# Autodesk Inventor assembly: Printer Assembly
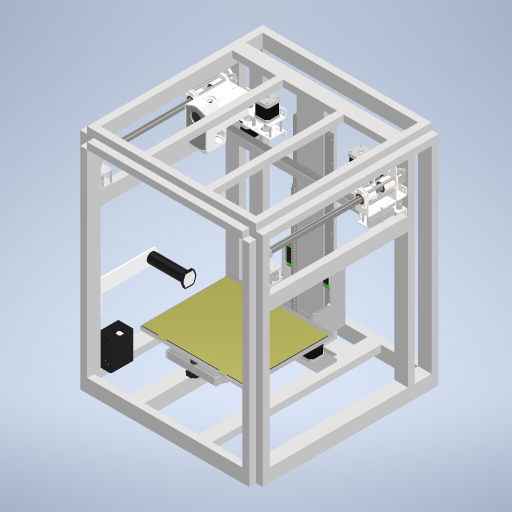
[picture p0: Inventor's stored thumbnail of the model, 512x512]
Saved by Autodesk Inventor 2024 (Build 280153000, 153)
## iProperties
Created: 2024-12-15
Part Number: Printer Assembly
Document SubType Name: Assembly
Designer: Ishaan
Author: Ishaan
## Documents named in this file (6)
- E:\Projects\Axiom--IDEX-3D-Printer\CAD\Printer Assembly.iam
- E:\Projects\Axiom--IDEX-3D-Printer\CAD\Rev V Envelope Frame Study.ipt
- E:\Projects\Axiom--IDEX-3D-Printer\CAD\04 - Gantry\Static Gantry Assembly.iam
- E:\Projects\Axiom--IDEX-3D-Printer\CAD\02 - Z-axis\R2 Z-axis Assembly.iam
- E:\Projects\Axiom--IDEX-3D-Printer\CAD\04 - Gantry\Gantry Assembly.iam
- E:\Projects\Axiom--IDEX-3D-Printer\CAD\06 - Filament Path\Filament Path Assembly.iam
## Components (5 placed, 5 different names)
1. Rev V Envelope Frame Study:1 — Flush:1, Flush:2, Flush:3, Flush:4, Flush:5, Flush:6, Flush:7, Flush:8, Flush:9
2. Static Gantry Assembly:1 [sub-assembly] — Flush:1, Flush:2, Flush:3, Mate:1, Mate:2, Mate:3, Mate:4
3. R2 Z-axis Assembly:1 [sub-assembly] — Flush:4, Flush:5, Flush:6
4. Gantry Assembly:1 [sub-assembly] — Mate:1, Mate:2, Mate:3, Mate:4
5. Filament Path Assembly:1 [sub-assembly] — Flush:7, Flush:8, Flush:9
## Relationships (13: Flush 9, Mate 4)
- Flush:1: Rev V Envelope Frame Study:1 ↔ Static Gantry Assembly:1
- Flush:2: Rev V Envelope Frame Study:1 ↔ Static Gantry Assembly:1
- Flush:3: Rev V Envelope Frame Study:1 ↔ Static Gantry Assembly:1
- Flush:4: Rev V Envelope Frame Study:1 ↔ R2 Z-axis Assembly:1
- Flush:5: Rev V Envelope Frame Study:1 ↔ R2 Z-axis Assembly:1
- Flush:6: Rev V Envelope Frame Study:1 ↔ R2 Z-axis Assembly:1
- Flush:7: Rev V Envelope Frame Study:1 ↔ Filament Path Assembly:1
- Flush:8: Rev V Envelope Frame Study:1 ↔ Filament Path Assembly:1
- Flush:9: Rev V Envelope Frame Study:1 ↔ Filament Path Assembly:1
- Mate:1: Static Gantry Assembly:1 ↔ Gantry Assembly:1
- Mate:2: Static Gantry Assembly:1 ↔ Gantry Assembly:1
- Mate:3 (1 mm): Static Gantry Assembly:1 ↔ Gantry Assembly:1
- Mate:4 (1 mm): Static Gantry Assembly:1 ↔ Gantry Assembly:1
